# Autodesk Inventor assembly: test_assembly
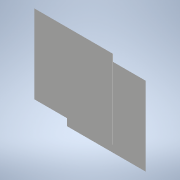
[picture p0: Inventor's stored thumbnail of the model, 180x180]
Saved by Autodesk Inventor 2021 (Build 250183000, 183)
## iProperties
Created: 2020-08-05
Part Number: test_assembly
Document SubType Name: Assembly
Designer: aydan
Author: aydan
## Documents named in this file (2)
- C:\Users\aydan\Documents\Inventor\Garcia_Lab\CAD_Models\test_assembly.iam
- C:\Users\aydan\Documents\Inventor\Garcia_Lab\CAD_Models\electrode.ipt
## Components (2 placed, 1 different names)
1. electrode:1 — Mate:3
2. electrode:2 — Mate:3
## Relationships (1: Mate 1)
- Mate:3 (0.3 mm): electrode:1 ↔ electrode:2
